# Autodesk Inventor assembly: Ensamble_Llanta
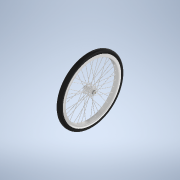
[picture p0: Inventor's stored thumbnail of the model, 180x180]
Saved by Autodesk Inventor 2021 (Build 250183000, 183)
## iProperties
Created: 2021-04-15
Part Number: Ensamble_Llanta
Document SubType Name: Assembly
Designer: j2seb
Author: j2seb
## Documents named in this file (8)
- C:\Git\Proyecto_APM\02 Inventor\bicicleta_ruta\otros\Ensamble_Llanta.iam
- C:\Git\Proyecto_APM\02 Inventor\bicicleta_ruta\otros\manzana1.ipt
- C:\Git\Proyecto_APM\02 Inventor\bicicleta_ruta\otros\protector.ipt
- C:\Git\Proyecto_APM\02 Inventor\bicicleta_ruta\otros\cubierta.ipt
- C:\Git\Proyecto_APM\02 Inventor\bicicleta_ruta\otros\neumatico.ipt
- C:\Git\Proyecto_APM\02 Inventor\bicicleta_ruta\otros\cinta_protectora.ipt
- C:\Git\Proyecto_APM\02 Inventor\bicicleta_ruta\otros\tuerca_manzana_1.ipt
- C:\Git\Proyecto_APM\02 Inventor\bicicleta_ruta\llanta_ruta_2.ipt
## Components (8 placed, 7 different names)
1. manzana1:1 — Coincidencia:1, Coincidencia:2, Coincidencia:3, Coincidencia:4
2. protector:1
3. cubierta:1
4. neumatico:1 — Nivelación:1
5. cinta_protectora:1 — Nivelación:2
6. tuerca_manzana_1:1 — Coincidencia:1, Coincidencia:4
7. tuerca_manzana_1:2 — Coincidencia:2, Coincidencia:3
8. llanta_ruta_2:1 — Flush:3
## Relationships (7: Mate 4, Flush 3)
- Nivelación:1 [Flush]: neumatico:1
- Nivelación:2 [Flush]: cinta_protectora:1
- Coincidencia:1 [Mate]: manzana1:1 ↔ tuerca_manzana_1:1
- Coincidencia:2 [Mate]: manzana1:1 ↔ tuerca_manzana_1:2
- Coincidencia:3 [Mate]: manzana1:1 ↔ tuerca_manzana_1:2
- Coincidencia:4 [Mate]: manzana1:1 ↔ tuerca_manzana_1:1
- Flush:3: llanta_ruta_2:1
